# Autodesk Inventor assembly: JibCrane
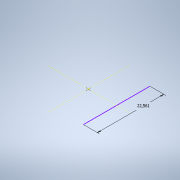
[picture p0: Inventor's stored thumbnail of the model, 180x180]
Saved by Autodesk Inventor 2022 (Build 260153000, 153)
## iProperties
Created: 2023-08-15
Part Number: JibCrane
Document SubType Name: Assembly
Designer: ASUS
Author: ASUS
## Documents named in this file (2)
- C:\Users\ASUS\Documents\Inventor\JibCrane\JibCrane.iam
- C:\Users\ASUS\Documents\Inventor\JibCrane\Columna.ipt
## Components (1 placed, 1 different names)
1. Columna:1
## Named parameters: Log_Col = 4749.8 mm, Log_Bra = 50.8 mm, Log_Viga = 1 mm, CD = 2540 mm, BC = 1473.2 mm, AB = 736.6 mm, BE = 1473.2 mm, EF0 = 2184.4 mm
